# Autodesk Inventor assembly: 0 ASY PRS MAIN
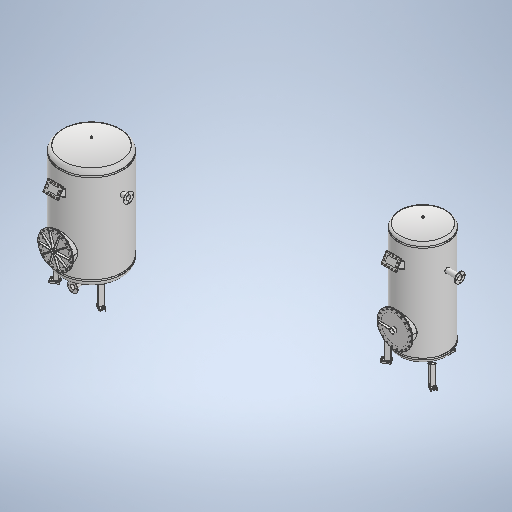
[picture p0: Inventor's stored thumbnail of the model, 512x512]
Saved by Autodesk Inventor 2026.2 (Build 302298000, 298)
## iProperties
Created: 2026-05-15
Part Number: 0 ASY PRS MAIN
Document SubType Name: Assembly
Designer: admin
Author: admin
## Documents named in this file (3)
- C:\Users\admin\Documents\Inventor\PRS-Purovsk\0 ASY PRS MAIN.iam
- C:\Users\admin\Documents\Inventor\PRS-Purovsk\ASY PRS 2 Filter column D1200.iam
- C:\Users\admin\Documents\Inventor\PRS-Purovsk\ASY PRS 2 Filter column D1200 940.iam
## Components (2 placed, 2 different names)
1. ASY PRS 2 Filter column D1200.iam:1 [sub-assembly] — Flush:2
2. ASY PRS 2 Filter column D1200 940:1 [sub-assembly]
## Relationships (1: Flush 1)
- Flush:2: ASY PRS 2 Filter column D1200.iam:1
